# Autodesk Inventor assembly: Main_assssembly
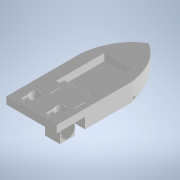
[picture p0: Inventor's stored thumbnail of the model, 180x180]
Saved by Autodesk Inventor 2020.1 (Build 241239000, 239)
## iProperties
Created: 2022-02-07
Part Number: Main_assssembly
Document SubType Name: Assembly
Designer: OEM
Author: OEM
## Documents named in this file (3)
- D:\Studia\Bobr\Repo\CAD\Main_assssembly.iam
- D:\Studia\Bobr\Repo\CAD\MainBody.ipt
- D:\Studia\Bobr\Repo\CAD\engine_connector_sleeve.ipt
## Components (2 placed, 2 different names)
1. MainBody:2 — Rotational:1
2. engine_connector_sleeve:1 — Rotational:1
## Relationships (1: RevoluteJoint 1)
- Rotational:1 [RevoluteJoint]: MainBody:2 ↔ engine_connector_sleeve:1
